# Autodesk Inventor assembly: Drum Assembly
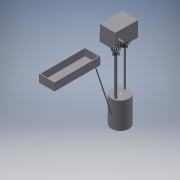
[picture p0: Inventor's stored thumbnail of the model, 180x180]
Saved by Autodesk Inventor 2019 (Build 230136000, 136)
## iProperties
Created: 2019-11-06
Part Number: Drum Assembly
Document SubType Name: Assembly
Designer: Administrator
Author: Administrator
## Documents named in this file (12)
- H:\Cad 30\Digestor parts so far 11.6\Drum Assembly.iam
- H:\Cad 30\Digestor parts so far 11.6\parts\Lid.ipt
- H:\Cad 30\Digestor parts so far 11.6\parts\Base.ipt
- H:\Cad 30\Digestor parts so far 11.6\Out pipe.ipt
- H:\Cad 30\Digestor parts so far 11.6\Trough.ipt
- H:\Cad 30\Digestor parts so far 11.6\Gas Hose.ipt
- H:\Cad 30\Digestor parts so far 11.6\Poop chute.ipt
- H:\Cad 30\Digestor parts so far 11.6\Funnel.ipt
- H:\Cad 30\Digestor parts so far 11.6\Gas to Gen pipe.ipt
- H:\Cad 30\Digestor parts so far 11.6\Gat to burner funnel.ipt
- H:\Cad 30\Digestor parts so far 11.6\Burner.ipt
- H:\Cad 30\Digestor parts so far 11.6\Generator.ipt
## Components (11 placed, 11 different names)
1. Lid:1 — Mate:2, Mate:3, Mate:5, Mate:10, Mate:11, Mate:12, Mate:15
2. Base:1 — Mate:1, Mate:4, Mate:5, Mate:6, Mate:7
3. Out pipe:1 — Mate:6, Mate:7, Mate:8, Mate:9
4. Trough:1 — Mate:8, Mate:9
5. Gas Hose:1 — Mate:10, Mate:11, Mate:21, Mate:22
6. Poop chute:1 — Mate:12, Mate:15, Mate:16, Mate:17, Mate:18
7. Funnel:1 — Mate:16, Mate:17, Mate:18
8. Gas to Gen pipe:1 — Mate:21, Mate:22, Flush:1, Mate:23, Mate:24
9. Gat to burner funnel:1 — Flush:1, Mate:23, Mate:24, Mate:25, Mate:26, Mate:28, Mate:30, Mate:32, Mate:33
10. Burner:1 — Mate:25, Mate:26, Mate:30, Mate:31
11. Generator:1 — Mate:32, Mate:33
## Relationships (29: Mate 28, Flush 1)
- Mate:1: Base:1
- Mate:2: Lid:1
- Mate:3: Lid:1
- Mate:4: Base:1
- Mate:5: Lid:1 ↔ Base:1
- Mate:6: Base:1 ↔ Out pipe:1
- Mate:7: Base:1 ↔ Out pipe:1
- Mate:8: Out pipe:1 ↔ Trough:1
- Mate:9: Out pipe:1 ↔ Trough:1
- Mate:10: Lid:1 ↔ Gas Hose:1
- Mate:11: Lid:1 ↔ Gas Hose:1
- Mate:12: Lid:1 ↔ Poop chute:1
- Mate:15: Lid:1 ↔ Poop chute:1
- Mate:16: Poop chute:1 ↔ Funnel:1
- Mate:17: Poop chute:1 ↔ Funnel:1
- Mate:18: Poop chute:1 ↔ Funnel:1
- Mate:21: Gas Hose:1 ↔ Gas to Gen pipe:1
- Mate:22: Gas Hose:1 ↔ Gas to Gen pipe:1
- Flush:1: Gas to Gen pipe:1 ↔ Gat to burner funnel:1
- Mate:23: Gas to Gen pipe:1 ↔ Gat to burner funnel:1
- Mate:24: Gas to Gen pipe:1 ↔ Gat to burner funnel:1
- Mate:25: Gat to burner funnel:1 ↔ Burner:1
- Mate:26: Gat to burner funnel:1 ↔ Burner:1
- Mate:28: Gat to burner funnel:1
- Mate:29
- Mate:30: Gat to burner funnel:1 ↔ Burner:1
- Mate:31: Burner:1
- Mate:32: Gat to burner funnel:1 ↔ Generator:1
- Mate:33: Gat to burner funnel:1 ↔ Generator:1
